# Autodesk Inventor assembly: MultiPass325V_outsideIn
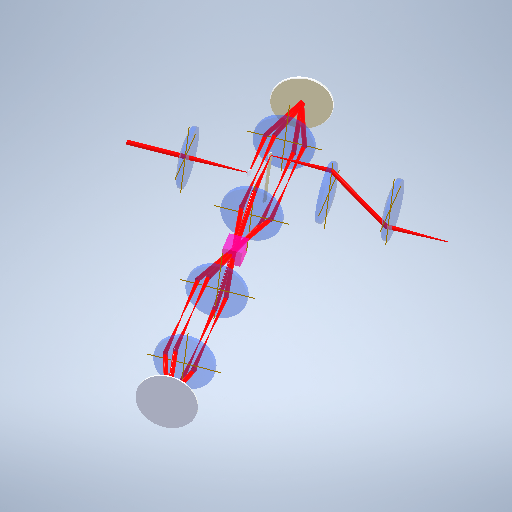
[picture p0: Inventor's stored thumbnail of the model, 512x512]
Saved by Autodesk Inventor 2026 (Build 300175050, 175E)
## iProperties
Created: 2024-08-19
Part Number: MultiPass325V_outsideIn
Document SubType Name: Assembly
Designer: User
Author: User
## Documents named in this file (14)
- C:\Users\newmanza\Documents\KerlinLab\Grants\EOD ROI 2025\MechanicalDrawingMultipass\MultiPass325V_outsideIn.iam
- C:\Users\newmanza\Documents\KerlinLab\Grants\EOD ROI 2025\MechanicalDrawingMultipass\BB1-E02-Solidworks.ipt
- C:\Users\newmanza\Documents\KerlinLab\Grants\EOD ROI 2025\MechanicalDrawingMultipass\LA1608-AB-Solidworks\LA1608-AB-Solidworks.ipt
- C:\Users\newmanza\Documents\KerlinLab\Grants\EOD ROI 2025\MechanicalDrawingMultipass\LaserBeamEntry1.ipt
- C:\Users\newmanza\Documents\KerlinLab\Grants\EOD ROI 2025\MechanicalDrawingMultipass\EntryMirror.ipt
- C:\Users\newmanza\Documents\KerlinLab\Grants\EOD ROI 2025\MechanicalDrawingMultipass\ExitMirror.ipt
- C:\Users\newmanza\Documents\KerlinLab\Grants\EOD ROI 2025\MechanicalDrawingMultipass\LaserBeamEntry2.ipt
- C:\Users\newmanza\Documents\KerlinLab\Grants\EOD ROI 2025\MechanicalDrawingMultipass\LaserBeamCenter1.ipt
- C:\Users\newmanza\Documents\KerlinLab\Grants\EOD ROI 2025\MechanicalDrawingMultipass\LaserBeamMirrorAngle1.ipt
- C:\Users\newmanza\Documents\KerlinLab\Grants\EOD ROI 2025\MechanicalDrawingMultipass\LaserBeamCenter2.ipt
- C:\Users\newmanza\Documents\KerlinLab\Grants\EOD ROI 2025\MechanicalDrawingMultipass\LaserBeamMirrorAngle2.ipt
- C:\Users\newmanza\Documents\KerlinLab\Grants\EOD ROI 2025\MechanicalDrawingMultipass\KTN1.ipt
- C:\Users\newmanza\Documents\KerlinLab\Grants\EOD ROI 2025\MechanicalDrawingMultipass\LoopPlane1.ipt
- C:\Users\newmanza\Documents\KerlinLab\Grants\EOD ROI 2025\MechanicalDrawingMultipass\LaserBeamFinal.ipt
## Components (46 placed, 13 different names)
1. BB1-E02-Solidworks:1 — Mate:15, Mate:16, Mate:17, Mate:115, Mate:116
2. BB1-E02-Solidworks:2 — Mate:13, Mate:14, Mate:18
3. LA1608-AB-Solidworks:1 — Mate:5, Mate:6, Mate:7, Mate:8, Mate:11, Mate:12, Mate:45, Mate:56, Mate:86, Mate:88, Mate:106
4. LA1608-AB-Solidworks:3 — Mate:27, Mate:28
5. LA1608-AB-Solidworks:4 — Mate:7, Mate:8, Mate:12, Mate:13, Mate:14, Mate:18
6. LA1608-AB-Solidworks:5 — Mate:3, Mate:4, Mate:5, Mate:6, Mate:10, Mate:11, Mate:21, Mate:44, Mate:57, Mate:87, Mate:89, Mate:104, Mate:105
7. LA1608-AB-Solidworks:6 — Mate:3, Mate:4, Mate:10, Mate:15, Mate:16, Mate:17, Mate:19, Mate:20, Flush:1, Mate:75, Mate:84
8. LA1608-AB-Solidworks:7 — Mate:29, Flush:2
9. LaserBeamEntry1:2
10. EntryMirror:1
11. LaserBeamEntry2:1
12. LaserBeamEntry2:2
13. LaserBeamEntry2:3
14. LaserBeamEntry2:4
15. LaserBeamCenter1:1
16. LaserBeamEntry2:5
17. LaserBeamEntry2:6
18. LaserBeamEntry2:8
19. LaserBeamEntry2:9
20. LaserBeamEntry2:10
21. LaserBeamCenter1:2
22. LaserBeamEntry2:11
23. LaserBeamMirrorAngle1:1
24. LaserBeamMirrorAngle1:2
25. LaserBeamMirrorAngle1:3
26. LaserBeamEntry2:12
27. LaserBeamEntry2:13
28. LaserBeamEntry2:14
29. LaserBeamEntry2:15 — Mate:75, Mate:84
30. LaserBeamEntry2:16
31. LaserBeamEntry2:17
32. LaserBeamEntry2:18
33. LaserBeamCenter2:1
34. LaserBeamCenter2:2
35. LaserBeamEntry2:19 — Mate:119
36. ExitMirror:2
37. LaserBeamMirrorAngle2:1
38. LaserBeamMirrorAngle2:2
39. KTN1:1 — Mate:104, Mate:105, Mate:106, Mate:114
40. LoopPlane1:1 — Mate:113, Mate:114
41. LaserBeamMirrorAngle2:3 — Mate:115, Mate:116
42. LaserBeamMirrorAngle1:4
43. LA1608-AB-Solidworks:9
44. LaserBeamEntry1:3
45. LaserBeamEntry2:20
46. LaserBeamFinal:1
## Relationships (45: Mate 43, Flush 2)
- Mate:3: LA1608-AB-Solidworks:5 ↔ LA1608-AB-Solidworks:6
- Mate:4 (-50 mm): LA1608-AB-Solidworks:5 ↔ LA1608-AB-Solidworks:6
- Mate:5: LA1608-AB-Solidworks:1 ↔ LA1608-AB-Solidworks:5
- Mate:6 (50 mm): LA1608-AB-Solidworks:1 ↔ LA1608-AB-Solidworks:5
- Mate:7: LA1608-AB-Solidworks:1 ↔ LA1608-AB-Solidworks:4
- Mate:8 (-50 mm): LA1608-AB-Solidworks:1 ↔ LA1608-AB-Solidworks:4
- Mate:10: LA1608-AB-Solidworks:5 ↔ LA1608-AB-Solidworks:6
- Mate:11: LA1608-AB-Solidworks:1 ↔ LA1608-AB-Solidworks:5
- Mate:12: LA1608-AB-Solidworks:1 ↔ LA1608-AB-Solidworks:4
- Mate:13: BB1-E02-Solidworks:2 ↔ LA1608-AB-Solidworks:4
- Mate:14 (25 mm): BB1-E02-Solidworks:2 ↔ LA1608-AB-Solidworks:4
- Mate:15: BB1-E02-Solidworks:1 ↔ LA1608-AB-Solidworks:6
- Mate:16 (-25 mm): BB1-E02-Solidworks:1 ↔ LA1608-AB-Solidworks:6
- Mate:17: BB1-E02-Solidworks:1 ↔ LA1608-AB-Solidworks:6
- Mate:18: BB1-E02-Solidworks:2 ↔ LA1608-AB-Solidworks:4
- Mate:19: LA1608-AB-Solidworks:6
- Mate:20: LA1608-AB-Solidworks:6
- Mate:21: LA1608-AB-Solidworks:5
- Mate:22
- Mate:23
- Flush:1 (-25 mm): LA1608-AB-Solidworks:6
- Mate:24
- Mate:25
- Mate:27: LA1608-AB-Solidworks:3
- Mate:28 (-34 mm): LA1608-AB-Solidworks:3
- Mate:29: LA1608-AB-Solidworks:7
- Flush:2 (-25 mm): LA1608-AB-Solidworks:7
- Mate:44: LA1608-AB-Solidworks:5
- Mate:45: LA1608-AB-Solidworks:1
- Mate:56: LA1608-AB-Solidworks:1
- Mate:57: LA1608-AB-Solidworks:5
- Mate:75: LA1608-AB-Solidworks:6 ↔ LaserBeamEntry2:15
- Mate:84: LA1608-AB-Solidworks:6 ↔ LaserBeamEntry2:15
- Mate:86: LA1608-AB-Solidworks:1
- Mate:87: LA1608-AB-Solidworks:5
- Mate:88: LA1608-AB-Solidworks:1
- Mate:89: LA1608-AB-Solidworks:5
- Mate:104: LA1608-AB-Solidworks:5 ↔ KTN1:1
- Mate:105 (25 mm): LA1608-AB-Solidworks:5 ↔ KTN1:1
- Mate:106: LA1608-AB-Solidworks:1 ↔ KTN1:1
- Mate:113: LoopPlane1:1
- Mate:114: KTN1:1 ↔ LoopPlane1:1
- Mate:115: BB1-E02-Solidworks:1 ↔ LaserBeamMirrorAngle2:3
- Mate:116: BB1-E02-Solidworks:1 ↔ LaserBeamMirrorAngle2:3
- Mate:119: LaserBeamEntry2:19
